# Autodesk Inventor assembly: Anode
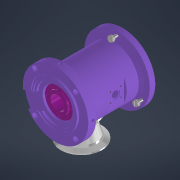
[picture p0: Inventor's stored thumbnail of the model, 180x180]
Saved by Autodesk Inventor 2022 (Build 260153000, 153)
## iProperties
Created: 2022-03-30
Part Number: Anode
Document SubType Name: Assembly
Designer: Vinicius Miguel
Author: Vinicius Miguel
## Documents named in this file (6)
- C:\ViniFiles\SEM-Mechanical\Anode.iam
- C:\ViniFiles\SEM-Mechanical\012.ipt
- C:\ViniFiles\SEM-Mechanical\013.ipt
- C:\ViniFiles\SEM-Mechanical\014.ipt
- C:\ViniFiles\SEM-Mechanical\015.ipt
- C:\ViniFiles\SEM-Mechanical\024.ipt
## Components (7 placed, 5 different names)
1. 012:1 — Mate:1, Flush:1, Flush:2, Mate:2, Mate:4, Rotational:2, Mate:5, Rotational:3, Rotational:4, Rotational:5
2. 013:1 — Mate:2, Mate:3, Mate:4, Rotational:1
3. 014:1 — Rotational:2, Mate:5
4. 015:1 — Rotational:1
5. 024:1 — Rotational:5
6. 024:2 — Rotational:3
7. 024:3 — Rotational:4
## Relationships (12: Mate 5, RevoluteJoint 5, Flush 2)
- Mate:1: 012:1
- Flush:1: 012:1
- Flush:2: 012:1
- Mate:2: 012:1 ↔ 013:1
- Mate:3: 013:1
- Mate:4: 012:1 ↔ 013:1
- Rotational:1 [RevoluteJoint]: 013:1 ↔ 015:1
- Rotational:2 [RevoluteJoint]: 012:1 ↔ 014:1
- Mate:5: 012:1 ↔ 014:1
- Rotational:3 [RevoluteJoint]: 012:1 ↔ 024:2
- Rotational:4 [RevoluteJoint]: 012:1 ↔ 024:3
- Rotational:5 [RevoluteJoint]: 012:1 ↔ 024:1
